# Autodesk Inventor assembly: RearLowerAArmandBracket
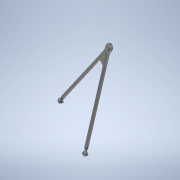
[picture p0: Inventor's stored thumbnail of the model, 180x180]
Saved by Autodesk Inventor 2021 (Build 250183000, 183)
## iProperties
Created: 2019-09-17
Part Number: RearLowerAArmandBracket
Document SubType Name: Assembly
Designer: beckerdj
Author: beckerdj
## Documents named in this file (10)
- C:\Users\cooks\Downloads\RearLowerAArmandBracket.iam
- C:\Users\cooks\Downloads\Weld Cup Model.ipt
- C:\Users\cooks\Downloads\LowControlArmPlateTabF.ipt
- C:\Users\cooks\Downloads\LowAArmTubeF.ipt
- C:\Users\cooks\Downloads\60645K131_STEEL BALL JOINT ROD END.ipt
- C:\Users\cooks\Downloads\Weldable Tube End.ipt
- C:\Users\cooks\Downloads\63195K670_STEEL BALL JOINT SWIVEL BEARING.ipt
- C:\Users\cooks\Downloads\FinalFrontLowerPlate.ipt
- C:\Users\cooks\Downloads\RIGHT BRACKET ARM FLAT (1).ipt
- C:\Users\cooks\Downloads\Bushings_MC_Mounting.ipt
## Components (15 placed, 9 different names)
1. Weld Cup Model:1 — Insert:5, Mate:1, Flush:1
2. LowControlArmPlateTabF:1 — Mate:9, Mate:10, Mate:11
3. LowControlArmPlateTabF:2 — Mate:6, Mate:7, Mate:8
4. LowAArmTubeF:1 — Insert:1, Mate:4, Mate:5, Tangent:1
5. LowAArmTubeF:2 — Insert:2, Mate:2, Mate:3, Tangent:2
6. 60645K131_STEEL BALL JOINT ROD END:1 — Insert:3, Mate:13
7. 60645K131_STEEL BALL JOINT ROD END:2 — Insert:4, Mate:12
8. Weldable Tube End:1 — Insert:1, Insert:4
9. Weldable Tube End:2 — Insert:2, Insert:3
10. 63195K670_STEEL BALL JOINT SWIVEL BEARING:1 — Insert:5
11. FinalFrontLowerPlate:1 — Mate:1, Flush:1, Mate:2, Mate:3, Mate:4, Mate:5, Mate:6, Mate:7, Mate:8, Mate:9, Mate:10, Mate:11, Tangent:1, Tangent:2
12. RIGHT BRACKET ARM FLAT (1):1 — Mate:12, Mate:14
13. RIGHT BRACKET ARM FLAT (1):2 — Mate:13, Mate:15
14. Bushings_MC_Mounting:1 — Mate:14
15. Bushings_MC_Mounting:2 — Mate:15
## Relationships (23: Mate 15, Insert 5, Tangent 2, Flush 1)
- Insert:1: LowAArmTubeF:1 ↔ Weldable Tube End:1
- Insert:2: LowAArmTubeF:2 ↔ Weldable Tube End:2
- Insert:3: 60645K131_STEEL BALL JOINT ROD END:1 ↔ Weldable Tube End:2
- Insert:4: 60645K131_STEEL BALL JOINT ROD END:2 ↔ Weldable Tube End:1
- Insert:5: Weld Cup Model:1 ↔ 63195K670_STEEL BALL JOINT SWIVEL BEARING:1
- Mate:1: Weld Cup Model:1 ↔ FinalFrontLowerPlate:1
- Flush:1 (-4.7244 mm): Weld Cup Model:1 ↔ FinalFrontLowerPlate:1
- Mate:2: LowAArmTubeF:2 ↔ FinalFrontLowerPlate:1
- Mate:3: LowAArmTubeF:2 ↔ FinalFrontLowerPlate:1
- Mate:4: LowAArmTubeF:1 ↔ FinalFrontLowerPlate:1
- Mate:5: LowAArmTubeF:1 ↔ FinalFrontLowerPlate:1
- Mate:6: LowControlArmPlateTabF:2 ↔ FinalFrontLowerPlate:1
- Mate:7: LowControlArmPlateTabF:2 ↔ FinalFrontLowerPlate:1
- Mate:8: LowControlArmPlateTabF:2 ↔ FinalFrontLowerPlate:1
- Mate:9: LowControlArmPlateTabF:1 ↔ FinalFrontLowerPlate:1
- Mate:10: LowControlArmPlateTabF:1 ↔ FinalFrontLowerPlate:1
- Mate:11: LowControlArmPlateTabF:1 ↔ FinalFrontLowerPlate:1
- Tangent:1 (0.762 mm): LowAArmTubeF:1 ↔ FinalFrontLowerPlate:1
- Tangent:2 (0.762 mm): LowAArmTubeF:2 ↔ FinalFrontLowerPlate:1
- Mate:12: 60645K131_STEEL BALL JOINT ROD END:2 ↔ RIGHT BRACKET ARM FLAT (1):1
- Mate:13: 60645K131_STEEL BALL JOINT ROD END:1 ↔ RIGHT BRACKET ARM FLAT (1):2
- Mate:14: RIGHT BRACKET ARM FLAT (1):1 ↔ Bushings_MC_Mounting:1
- Mate:15: RIGHT BRACKET ARM FLAT (1):2 ↔ Bushings_MC_Mounting:2
